# Autodesk Inventor assembly: Conveyor Assembly
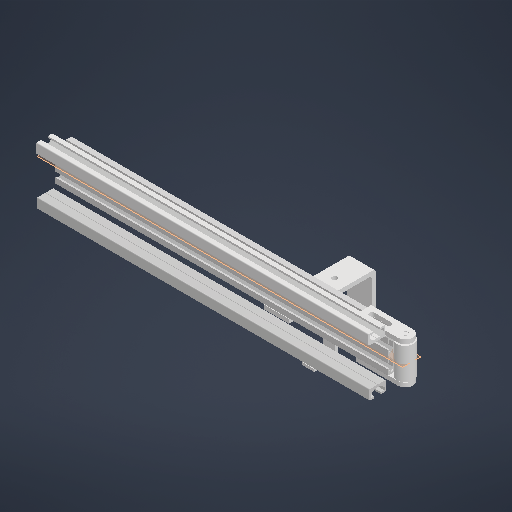
[picture p0: Inventor's stored thumbnail of the model, 512x512]
Saved by Autodesk Inventor 2027 (Build 310192000, 192)
## iProperties
Created: 2026-07-15
Part Number: Conveyor Assembly
Document SubType Name: Assembly
Designer: ratik
Author: ratik
## Documents named in this file (8)
- C:\Users\ratik\OneDrive\Personal Folder\00_Startup\00_MectoSYS_Repo\01_Mechanical_Design\01_CAD Design\3D file\03_Conveyor Assembly\Conveyor 2.0\Conveyor Assembly.iam
- C:\Users\ratik\OneDrive\Personal Folder\00_Startup\01_Mectosys_Prototype\01_Prototype\01_Mechanical\3D file\05_Pick and place\10_HFS5-2040-1500_Inventor\HFS5-2040-1500.ipt
- C:\Users\ratik\OneDrive\Personal Folder\00_Startup\00_MectoSYS_Repo\01_Mechanical_Design\01_CAD Design\3D file\03_Conveyor Assembly\Conveyor 2.0\roller bracket.ipt
- C:\Users\ratik\OneDrive\Personal Folder\00_Startup\00_MectoSYS_Repo\01_Mechanical_Design\01_CAD Design\3D file\03_Conveyor Assembly\Conveyor 2.0\roller.ipt
- C:\Users\ratik\OneDrive\Personal Folder\00_Startup\01_Mectosys_Prototype\01_Prototype\01_Mechanical\3D file\02_Slider\08_HFSPURE6-1220-2500_STEP_AP214_20260415\HFSPURE6-1220-2500\HFSPURE6-1220-2500.ipt
- C:\Users\ratik\OneDrive\Personal Folder\00_Startup\01_Mectosys_Prototype\01_Prototype\01_Mechanical\3D file\02_Slider\08_HFSPURE6-1220-2500_STEP_AP214_20260415\HFSPURE6-1220-2500\HFSPURE6-1220-2500_MIR1.ipt
- C:\Users\ratik\OneDrive\Personal Folder\00_Startup\00_MectoSYS_Repo\01_Mechanical_Design\01_CAD Design\3D file\03_Conveyor Assembly\Conveyor 2.0\Side holding bracket.ipt
- C:\Users\ratik\OneDrive\Personal Folder\00_Startup\00_MectoSYS_Repo\01_Mechanical_Design\01_CAD Design\3D file\03_Conveyor Assembly\Conveyor 2.0\Mounting Bracket.ipt
## Components (8 placed, 7 different names)
1. HFS5-2040-1500:1 — Mate:1, Flush:1, Mate:2, Flush:2, Mate:4, Mate:5, Flush:5, Mate:6, Mate:7, Mate:8, Mate:10, Flush:7
2. roller bracket:1 — Mate:1, Flush:1, Flush:3, Flush:4, Mate:3
3. roller bracket:2 — Mate:2, Flush:2, Flush:3
4. roller:1 — Flush:4, Mate:3
5. HFSPURE6-1220-2500:1 — Mate:4, Mate:5, Flush:5, Mate:9, Flush:6
6. HFSPURE6-1220-2500_MIR1:1
7. Side holding bracket:1 — Mate:9, Flush:6
8. Mounting Bracket:1 — Mate:10, Flush:7
## Relationships (17: Mate 10, Flush 7)
- Mate:1: HFS5-2040-1500:1 ↔ roller bracket:1
- Flush:1 (1 mm): HFS5-2040-1500:1 ↔ roller bracket:1
- Mate:2: HFS5-2040-1500:1 ↔ roller bracket:2
- Flush:2 (1 mm): HFS5-2040-1500:1 ↔ roller bracket:2
- Flush:3: roller bracket:1 ↔ roller bracket:2
- Flush:4: roller bracket:1 ↔ roller:1
- Mate:3: roller bracket:1 ↔ roller:1
- Mate:4 (2 mm): HFS5-2040-1500:1 ↔ HFSPURE6-1220-2500:1
- Mate:5 (3 mm): HFS5-2040-1500:1 ↔ HFSPURE6-1220-2500:1
- Flush:5: HFS5-2040-1500:1 ↔ HFSPURE6-1220-2500:1
- Mate:6: HFS5-2040-1500:1
- Mate:7: HFS5-2040-1500:1
- Mate:8: HFS5-2040-1500:1
- Mate:9: HFSPURE6-1220-2500:1 ↔ Side holding bracket:1
- Flush:6: HFSPURE6-1220-2500:1 ↔ Side holding bracket:1
- Mate:10: HFS5-2040-1500:1 ↔ Mounting Bracket:1
- Flush:7: HFS5-2040-1500:1 ↔ Mounting Bracket:1
